# Autodesk Inventor assembly: Rocker-Bogie-Robot-ASM-01
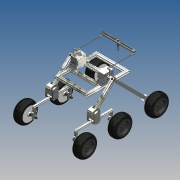
[picture p0: Inventor's stored thumbnail of the model, 180x180]
Saved by Autodesk Inventor 2018.2 (Build 222227000, 227)
## iProperties
Manager: feesmrt
Company: FRANC0R
Created: 2017-12-16
Part Number: Rocker-Bogie-Robot-ASM-01
Material: Generisch
Document SubType Name: Assembly
Designer: feesmrt
Project: Rescue Robot
Cost Center: -
Description: Rocker Bogie Robot Ver 01
Engineer: feesmrt
Authority: feesmrt
Stock Number: Rocker-Bogie-Robot-ASM-01
Author: feesmrt
Title: Rocker Bogie Robot Ver 01
Subject: Rescue Robot
Revision Number: 1
## Documents named in this file (5)
- D:\Programmierung\FRANC0R\CAD\02-Rocker-Bogie-Robot\Rocker-Bogie-Robot-ASM-01.iam
- D:\Programmierung\FRANC0R\CAD\02-Rocker-Bogie-Robot\100-CHASSIS\100-CHASSIS-ASM-01.iam
- D:\Programmierung\FRANC0R\CAD\02-Rocker-Bogie-Robot\200-ROCKER-BOGIE\200-ROCKER-BOGIE-ASM-01.iam
- D:\Programmierung\FRANC0R\CAD\02-Rocker-Bogie-Robot\200-ROCKER-BOGIE\200-ROCKER-BOGIE-ASM-02.iam
- D:\Programmierung\FRANC0R\CAD\02-Rocker-Bogie-Robot\200-ROCKER-BOGIE\200-60-DIFFERENTIAL\200-60-DIFFERENTIAL-CONNECTOR-01.iam
## Components (4 placed, 4 different names)
1. 100-CHASSIS-ASM-01:1 [sub-assembly] — Fluchtend:1, Fluchtend:2, Passend:1, Passend:2, Fluchtend:3
2. 200-ROCKER-BOGIE-ASM-01:1 [sub-assembly] — Fluchtend:1, Fluchtend:2, Passend:1, Passend:3, Passend:5, Passend:6
3. 200-ROCKER-BOGIE-ASM-02:1 [sub-assembly] — Passend:2, Passend:3, Fluchtend:3, Passend:4
4. 200-60-DIFFERENTIAL-CONNECTOR-01:1 [sub-assembly] — Passend:4, Passend:5, Passend:6
## Relationships (9: Mate 6, Flush 3)
- Fluchtend:1 [Flush]: 100-CHASSIS-ASM-01:1 ↔ 200-ROCKER-BOGIE-ASM-01:1
- Fluchtend:2 [Flush]: 100-CHASSIS-ASM-01:1 ↔ 200-ROCKER-BOGIE-ASM-01:1
- Passend:1 [Mate]: 100-CHASSIS-ASM-01:1 ↔ 200-ROCKER-BOGIE-ASM-01:1
- Passend:2 [Mate]: 100-CHASSIS-ASM-01:1 ↔ 200-ROCKER-BOGIE-ASM-02:1
- Passend:3 [Mate]: 200-ROCKER-BOGIE-ASM-01:1 ↔ 200-ROCKER-BOGIE-ASM-02:1
- Fluchtend:3 [Flush]: 100-CHASSIS-ASM-01:1 ↔ 200-ROCKER-BOGIE-ASM-02:1
- Passend:4 [Mate]: 200-ROCKER-BOGIE-ASM-02:1 ↔ 200-60-DIFFERENTIAL-CONNECTOR-01:1
- Passend:5 [Mate]: 200-ROCKER-BOGIE-ASM-01:1 ↔ 200-60-DIFFERENTIAL-CONNECTOR-01:1
- Passend:6 [Mate]: 200-ROCKER-BOGIE-ASM-01:1 ↔ 200-60-DIFFERENTIAL-CONNECTOR-01:1
